# Autodesk Inventor assembly: Arena assembly
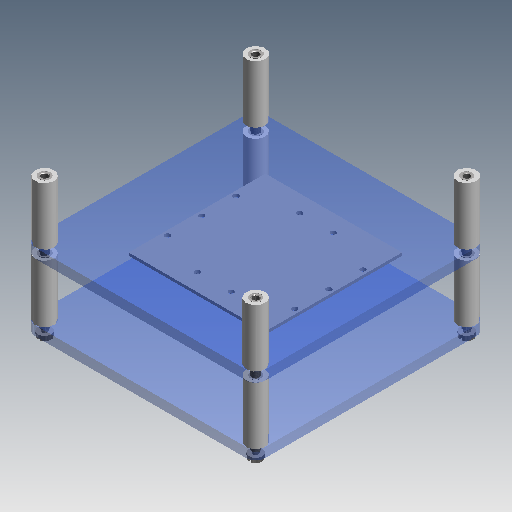
[picture p0: Inventor's stored thumbnail of the model, 512x512]
Saved by Autodesk Inventor 2020 (Build 240168000, 168)
## iProperties
Created: 2020-08-17
Part Number: Arena assembly
Document SubType Name: Assembly
Designer: ferrerx
Author: ferrerx
## Documents named in this file (7)
- C:\Users\ferrerx\Desktop\Prieto-Godino Lab\Drosophila Larvae Behavioural Device\Device design V3\Inventor Assembly\Arena assembly.iam
- C:\Users\ferrerx\Desktop\Prieto-Godino Lab\Drosophila Larvae Behavioural Device\Device design V3\Inventor Assembly\Arena.ipt
- C:\Users\ferrerx\Desktop\Prieto-Godino Lab\Drosophila Larvae Behavioural Device\Device design V3\Inventor Assembly\Arena spacer.ipt
- C:\Users\ferrerx\Desktop\Prieto-Godino Lab\Drosophila Larvae Behavioural Device\Device design V3\Inventor Assembly\LED Matrix 8X8.ipt
- C:\Users\ferrerx\Documents\Inventor\Content Center Files\R2020\en-US\AS 1427(10)\AS 1427 - M4 x 16(7).ipt
- C:\Users\ferrerx\Documents\Inventor\Content Center Files\R2020\en-US\DIN 976-1 B\DIN 976-1 - M4 x 20 - B.ipt
- C:\Users\ferrerx\Documents\Inventor\Content Center Files\R2020\en-US\GB 809-88 A\Nut GB 809 A M4 x 4.ipt
## Components (35 placed, 6 different names)
1. Arena:1 — Mate:176, Mate:177, Mate:178, Mate:241, Mate:242, Mate:255, Mate:256, Mate:257, Mate:258, Mate:259, Mate:260, Mate:261, Mate:262, Mate:271
2. Arena spacer:1 — Mate:177, Mate:178, Mate:313, Mate:316, Mate:326, Mate:328
3. Arena spacer:2 — Mate:176, Mate:312, Mate:315, Mate:322, Mate:325
4. Arena spacer:3 — Mate:242, Mate:317, Mate:332, Mate:333
5. Arena spacer:4 — Mate:241, Mate:314, Mate:318, Flush:1, Mate:319
6. Arena spacer:5 — Mate:258, Mate:261, Mate:264, Mate:265, Mate:320, Mate:321
7. Arena spacer:6 — Mate:256, Mate:260, Mate:263, Mate:312, Mate:323, Mate:324
8. Arena spacer:7 — Mate:255, Mate:259, Mate:313, Mate:327, Mate:329
9. Arena spacer:8 — Mate:257, Mate:262, Mate:330, Mate:331
10. Arena:2 — Mate:263, Mate:264, Mate:265, Mate:304, Mate:305, Mate:306, Mate:307, Mate:308, Mate:309, Mate:310, Mate:311
11. LED Matrix 8X8:1 — Mate:271
12. AS 1427 (8) - Metric M4 x 16:11 — Mate:306, Mate:310
13. AS 1427 (8) - Metric M4 x 16:12 — Mate:307, Mate:311
14. AS 1427 (8) - Metric M4 x 16:13 — Mate:304, Mate:309
15. AS 1427 (8) - Metric M4 x 16:14 — Mate:305, Mate:308
16. DIN 976-1 B M4 x 20:1 — Mate:314
17. DIN 976-1 B M4 x 20:2 — Mate:315
18. DIN 976-1 B M4 x 20:3 — Mate:316
19. DIN 976-1 B M4 x 20:4 — Mate:317
20. Nut GB/T 809-1988 Type A M4x4:1 — Mate:327
21. Nut GB/T 809-1988 Type A M4x4:2 — Mate:329
22. Nut GB/T 809-1988 Type A M4x4:3 — Mate:319
23. Nut GB/T 809-1988 Type A M4x4:4 — Mate:320
24. Nut GB/T 809-1988 Type A M4x4:5 — Mate:322
25. Nut GB/T 809-1988 Type A M4x4:6 — Mate:326
26. Nut GB/T 809-1988 Type A M4x4:7 — Mate:323
27. Nut GB/T 809-1988 Type A M4x4:8 — Mate:325
28. Nut GB/T 809-1988 Type A M4x4:9 — Mate:324
29. Nut GB/T 809-1988 Type A M4x4:10 — Mate:328
30. Nut GB/T 809-1988 Type A M4x4:11 — Mate:321
31. Nut GB/T 809-1988 Type A M4x4:12 — Mate:318, Flush:1
32. Nut GB/T 809-1988 Type A M4x4:13 — Mate:330
33. Nut GB/T 809-1988 Type A M4x4:14 — Mate:331
34. Nut GB/T 809-1988 Type A M4x4:15 — Mate:333
35. Nut GB/T 809-1988 Type A M4x4:16 — Mate:332
## Relationships (48: Mate 47, Flush 1)
- Mate:176: Arena:1 ↔ Arena spacer:2
- Mate:177: Arena:1 ↔ Arena spacer:1
- Mate:178: Arena:1 ↔ Arena spacer:1
- Mate:241: Arena:1 ↔ Arena spacer:4
- Mate:242: Arena:1 ↔ Arena spacer:3
- Mate:255: Arena:1 ↔ Arena spacer:7
- Mate:256: Arena:1 ↔ Arena spacer:6
- Mate:257: Arena:1 ↔ Arena spacer:8
- Mate:258: Arena:1 ↔ Arena spacer:5
- Mate:259: Arena:1 ↔ Arena spacer:7
- Mate:260: Arena:1 ↔ Arena spacer:6
- Mate:261: Arena:1 ↔ Arena spacer:5
- Mate:262: Arena:1 ↔ Arena spacer:8
- Mate:263: Arena spacer:6 ↔ Arena:2
- Mate:264: Arena spacer:5 ↔ Arena:2
- Mate:265: Arena spacer:5 ↔ Arena:2
- Mate:271: Arena:1 ↔ LED Matrix 8X8:1
- Mate:304: Arena:2 ↔ AS 1427 (8) - Metric M4 x 16:13
- Mate:305: Arena:2 ↔ AS 1427 (8) - Metric M4 x 16:14
- Mate:306: Arena:2 ↔ AS 1427 (8) - Metric M4 x 16:11
- Mate:307: Arena:2 ↔ AS 1427 (8) - Metric M4 x 16:12
- Mate:308: Arena:2 ↔ AS 1427 (8) - Metric M4 x 16:14
- Mate:309: Arena:2 ↔ AS 1427 (8) - Metric M4 x 16:13
- Mate:310: Arena:2 ↔ AS 1427 (8) - Metric M4 x 16:11
- Mate:311: Arena:2 ↔ AS 1427 (8) - Metric M4 x 16:12
- Mate:312: Arena spacer:2 ↔ Arena spacer:6
- Mate:313: Arena spacer:1 ↔ Arena spacer:7
- Mate:314: Arena spacer:4 ↔ DIN 976-1 B M4 x 20:1
- Mate:315: Arena spacer:2 ↔ DIN 976-1 B M4 x 20:2
- Mate:316: Arena spacer:1 ↔ DIN 976-1 B M4 x 20:3
- Mate:317: Arena spacer:3 ↔ DIN 976-1 B M4 x 20:4
- Mate:318: Arena spacer:4 ↔ Nut GB/T 809-1988 Type A M4x4:12
- Flush:1: Arena spacer:4 ↔ Nut GB/T 809-1988 Type A M4x4:12
- Mate:319: Arena spacer:4 ↔ Nut GB/T 809-1988 Type A M4x4:3
- Mate:320: Arena spacer:5 ↔ Nut GB/T 809-1988 Type A M4x4:4
- Mate:321: Arena spacer:5 ↔ Nut GB/T 809-1988 Type A M4x4:11
- Mate:322: Arena spacer:2 ↔ Nut GB/T 809-1988 Type A M4x4:5
- Mate:323: Arena spacer:6 ↔ Nut GB/T 809-1988 Type A M4x4:7
- Mate:324: Arena spacer:6 ↔ Nut GB/T 809-1988 Type A M4x4:9
- Mate:325: Arena spacer:2 ↔ Nut GB/T 809-1988 Type A M4x4:8
- Mate:326: Arena spacer:1 ↔ Nut GB/T 809-1988 Type A M4x4:6
- Mate:327: Arena spacer:7 ↔ Nut GB/T 809-1988 Type A M4x4:1
- Mate:328: Arena spacer:1 ↔ Nut GB/T 809-1988 Type A M4x4:10
- Mate:329: Arena spacer:7 ↔ Nut GB/T 809-1988 Type A M4x4:2
- Mate:330: Arena spacer:8 ↔ Nut GB/T 809-1988 Type A M4x4:13
- Mate:331: Arena spacer:8 ↔ Nut GB/T 809-1988 Type A M4x4:14
- Mate:332: Arena spacer:3 ↔ Nut GB/T 809-1988 Type A M4x4:16
- Mate:333: Arena spacer:3 ↔ Nut GB/T 809-1988 Type A M4x4:15
